# Autodesk Inventor assembly: BGBFS6900DD-25
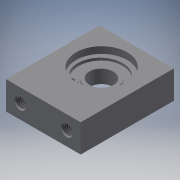
[picture p0: Inventor's stored thumbnail of the model, 180x180]
Saved by Autodesk Inventor 2019 (Build 230136000, 136)
## iProperties
Category: PARTsolutions
Company: MISUMI
Created: 2022-11-04
Part Number: BGBFS6900DD-25
Catalog Web Link: www.cadenas.de
Description: BGBFB, BGBF, BGBFA, BGBFSA, BGBFS-Bearings with Housings - Bottom Mount - h Configurable
Vendor: MISUMI
Document SubType Name: Assembly
Designer: psAdmin
Manufacturer: MISUMI
Mass: 12.4589 g
Surface Area: 65.3192 cm^2
Volume: 12.4589 cm^3
Density: 1 g/cm^3
Title: BGBFS6900DD-25
Author: Cadenas PARTsolutions
Comments: Bearings with Housings - Bottom Mount - h Configurable
PSOL_IDENT_0: {$CADENAS_DATA/23d-libs/misumi/metric/12_bearing_holders/bgbfb_asmtab.prj},247 {VTYP=3D},{STYP=ASSTA
PSOL_IDENT_1: B},{NB=BGBFS6900DD-25},{LINA=BGBFS6900DD-25},{NN=BGBFB, BGBF, BGBFA, BGBFSA, BGBFS},{DATE=18.09.2019
PSOL_IDENT_2: 08:29:03},{GEOMDATE=09.09.2019 09:38:45},{VERSION=},{LINEID=90},{WBVAR=MATB,MATH,STH,SEAL,HH,ALT1,A
PSOL_IDENT_3: LT2,ALT3},{WBNUMERIC=HH}  {NB=BGBFS6900DD-25},{LINA=BGBFS6900DD-25},{KT=DUMMY},{PN=BGBFS6900DD-25},{
PSOL_IDENT_4: TYPE=BGBFS},{MATB=SS},{MATBALG='S','Steel','SS','Stainless Steel'},{MATH=SUS304},{MATHALG='2017AA','
PSOL_IDENT_5: 2017 Aluminum Alloy','SUS304','304 Stainless Steel'},{STH=-},{STHALG='-','-'},{ARR=304 Stainless Ste
PSOL_IDENT_6: el},{ARR3D=-S},{BN=6900},{SEAL=DD},{SEALALG='ZZ','ZZ(Double Shielded)','VV','VV(Non-Contact Sealed R
PSOL_IDENT_7: ubber Seal)','DD','DD(Contact Sealed Rubber Seal)'},{HH=25},{HHALG=[25:50/1]},{DD=10},{D=22},{DDHH=1
PSOL_IDENT_8: 9},{B=6},{H=40},{H2=15},{L=32},{L1=20},{T=12},{M=M5},{M3D=5},{PITCH=0.8},{ALT1=},{KKC=0},{ALT2=},{MM=
PSOL_IDENT_9: 1.15},{DD2=23},{PPATH=bgbfb/bgbfb_asmtpl.prj},{ALT3=},{ALT1ALG= '', 'Bearing Assembled', '-NA', 'wit
PSOL_IDENT_10: h NA (Bearing not Assembled)' },{ALT2ALG= '','w/o KCC (C2 Chamfer)','-KCC','with KCC (C2 Chamfer)' }
PSOL_IDENT_11: ,{ALT3ALG= '','w/o KKC (C Chamfer)','-KKC','with KKC (C Chamfer)' }
NB: BGBFS6900DD-25
NN: BGBFB, BGBF, BGBFA, BGBFSA, BGBFS
NT: Bearings with Housings - Bottom Mount - h Configurable
NBSYN: $PN.
LINA: BGBFS6900DD-25
CATALOG: Misumi
PN: BGBFS6900DD-25
MATB: Stainless Steel
MATH: 304 Stainless Steel
STH: -
ARR: 304 Stainless Steel
BN: 6900
SEAL: DD(Contact Sealed Rubber Seal)
HH: 25
DD: 10
D: 22
DDHH: 19
B: 6
H: 40
L: 32
L1: 20
T: 12
M: M5
ALT1: Bearing Assembled
ALT2: w/o KCC (C2 Chamfer)
ALT3: w/o KKC (C Chamfer)
SUPPLIER: MISUMI
ARTICLENO: BGBFS6900DD-25
BOMINFO: BGBFS6900DD-25
CREATOR: CADENAS GmbH
## Documents named in this file (4)
- e:\temp\worker_COMMON_18\temp\tmp_5524_252_prE5O\format_0\BGBFS6900DD-25.iam
- e:\temp\worker_COMMON_18\temp\tmp_5524_252_prE5O\format_0\BGBFS6900DD-25-_h.ipt
- e:\temp\worker_COMMON_18\temp\tmp_5524_252_prE5O\format_0\bearing_6900.ipt
- e:\temp\worker_COMMON_18\temp\tmp_5524_252_prE5O\format_0\RRING-C-INT-S-22.ipt
## Components (3 placed, 3 different names)
1. BGBFS6900DD-25-_h:1 — to_bearing_XY@1 <-> to_housing_XY@2, to_bearing_Z@1 <-> to_housing_Z@2, to_bearing_YZ@1 <-> to_housing_YZ@2, to_ring_XY@1 <-> rr_XY@3, to_ring_Z@1 <-> rr_Z@3, to_ring_YZ@1 <-> rr_YZ@3
2. bearing_6900:1 — to_bearing_XY@1 <-> to_housing_XY@2, to_bearing_Z@1 <-> to_housing_Z@2, to_bearing_YZ@1 <-> to_housing_YZ@2
3. RRING-C-INT-S-22:1 — to_ring_XY@1 <-> rr_XY@3, to_ring_Z@1 <-> rr_Z@3, to_ring_YZ@1 <-> rr_YZ@3
## Relationships (6: Mate 4, Angle 2)
- to_bearing_XY@1 <-> to_housing_XY@2 [Mate]: BGBFS6900DD-25-_h:1 ↔ bearing_6900:1
- to_bearing_Z@1 <-> to_housing_Z@2 [Mate]: BGBFS6900DD-25-_h:1 ↔ bearing_6900:1
- to_bearing_YZ@1 <-> to_housing_YZ@2 [Angle] (0 deg): BGBFS6900DD-25-_h:1 ↔ bearing_6900:1
- to_ring_XY@1 <-> rr_XY@3 [Mate]: BGBFS6900DD-25-_h:1 ↔ RRING-C-INT-S-22:1
- to_ring_Z@1 <-> rr_Z@3 [Mate]: BGBFS6900DD-25-_h:1 ↔ RRING-C-INT-S-22:1
- to_ring_YZ@1 <-> rr_YZ@3 [Angle] (0 deg): BGBFS6900DD-25-_h:1 ↔ RRING-C-INT-S-22:1
